# Autodesk Inventor assembly: COXA
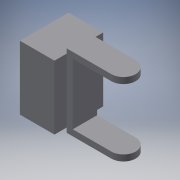
[picture p0: Inventor's stored thumbnail of the model, 180x180]
Saved by Autodesk Inventor 2017 (Build 210142000, 142)
## iProperties
Created: 2017-09-18
Part Number: COXA
Document SubType Name: Assembly
Designer: Alexander Miller
Author: Alexander Miller
## Documents named in this file (3)
- D:\Daten\Documents\Git\HeRo-Mini\Hardware\COXA.iam
- D:\Daten\Documents\Git\HeRo-Mini\Hardware\COXA_A.ipt
- D:\Daten\Documents\Git\HeRo-Mini\Hardware\COXA_B.ipt
## Components (2 placed, 2 different names)
1. COXA_A:1 — Rigid:1
2. COXA_B:1 — Rigid:1
## Relationships (1: WeldJoint 1)
- Rigid:1 [WeldJoint]: COXA_A:1 ↔ COXA_B:1
